# Autodesk Inventor assembly: XY_Assemblie
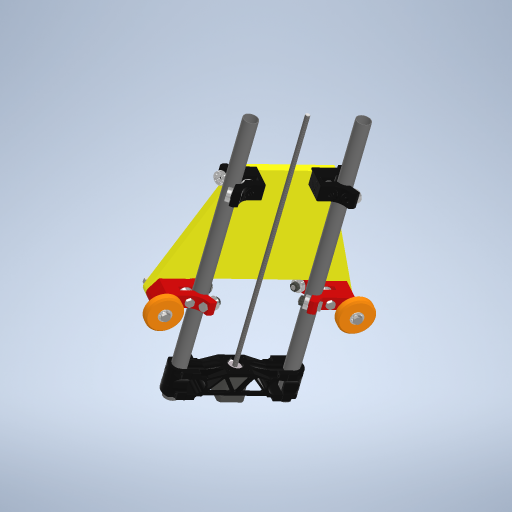
[picture p0: Inventor's stored thumbnail of the model, 512x512]
Saved by Autodesk Inventor 2023 (Build 270158000, 158)
## iProperties
Created: 2023-11-24
Part Number: XY_Assemblie
Document SubType Name: Assembly
Designer: danie
Author: danie
## Documents named in this file (14)
- D:\Diplomarbeit\3d-model\basis_roboter\low_rider_v2\custom_files\XY_Assemblie.iam
- D:\Diplomarbeit\3d-model\basis_roboter\low_rider_v2\custom_files\XZ.ipt
- D:\Diplomarbeit\3d-model\basis_roboter\low_rider_v2\custom_files\XZ_Pipe.ipt
- D:\Diplomarbeit\3d-model\basis_roboter\low_rider_v2\custom_files\XZ_Main.ipt
- D:\Diplomarbeit\3d-model\basis_roboter\low_rider_v2\custom_files\Lower_Za.ipt
- D:\Diplomarbeit\3d-model\basis_roboter\low_rider_v2\custom_files\Lower_Zb.ipt
- D:\Diplomarbeit\3d-model\basis_roboter\low_rider_v2\custom_files\Bearing.ipt
- D:\Diplomarbeit\3d-model\basis_roboter\low_rider_v2\custom_files\XY_Plate_.ipt
- D:\Diplomarbeit\3d-model\basis_roboter\low_rider_v2\custom_files\YZ_Roller_Assemblie.iam
- D:\Diplomarbeit\3d-model\basis_roboter\low_rider_v2\custom_files\Wheel_Assemblie.iam
- C:\Users\danie\OneDrive\Documents\Inventor\Content Center Files\R2023\en-US\AS 1111\AS 1111 - M8 x 70.ipt
- C:\Users\danie\OneDrive\Documents\Inventor\Content Center Files\R2023\en-US\ISO 4032(2)\ISO 4032 - M8 - ISO.ipt
- C:\Users\danie\OneDrive\Documents\Inventor\Content Center Files\R2023\en-US\AS 1111\AS 1111 - M8 x 90.ipt
- D:\Diplomarbeit\3d-model\basis_roboter\nema 17\dle-la-0003_01.ipt
## Components (31 placed, 13 different names)
1. XZ:1 — Rigid:20, Rigid:25
2. XZ_Pipe:1 — Rigid:25
3. XZ:2 — Rigid:19, Rigid:24
4. XZ_Pipe:2 — Rigid:24
5. XZ_Main:1 — Rigid:19, Rigid:20, Mate:17, Mate:19, Angle:3, Rigid:26
6. Lower_Za:1 — Rotational:3, Rotational:4, Rotational:5, Rigid:12
7. Lower_Zb:1 — Rotational:1, Rotational:2, Rigid:5, Rigid:13
8. Bearing:1 — Rotational:2
9. Bearing:2 — Rigid:5
10. Bearing:3 — Rotational:1
11. Bearing:4 — Rotational:3
12. Bearing:5 — Rotational:4
13. Bearing:6 — Rotational:5
14. XY_Plate_:1 — Rigid:12, Rigid:13, Angle:1, Rigid:22, Rigid:23, Mate:4, Mate:8, Mate:12, Mate:16, Mate:17, Mate:18, Angle:2
15. YZ_Roller_Assemblie:1 [sub-assembly] — Rigid:22, Mate:1, Mate:2, Mate:3, Rotational:15
16. YZ_Roller_Assemblie:2 [sub-assembly] — Rigid:23, Rotational:14, Mate:5, Mate:6, Mate:7
17. Wheel_Assemblie:1 [sub-assembly] — Rotational:15, Mate:9, Mate:10, Mate:11
18. Wheel_Assemblie:2 [sub-assembly] — Rotational:14, Mate:13, Mate:14, Mate:15
19. AS 1111 - Metric M8 x 70:1 — Mate:1, Mate:2
20. ISO 4032 M8:1 — Mate:3, Mate:4, Insert:1
21. ISO 4032 M8:2 — Insert:1
22. AS 1111 - Metric M8 x 70:2 — Mate:5, Mate:6
23. ISO 4032 M8:3 — Mate:7, Mate:8, Insert:2
24. ISO 4032 M8:4 — Insert:2
25. AS 1111 - Metric M8 x 90:1 — Mate:9, Mate:10
26. ISO 4032 M8:5 — Mate:11, Mate:12, Insert:3
27. ISO 4032 M8:6 — Insert:3
28. AS 1111 - Metric M8 x 90:2 — Mate:13, Mate:14
29. ISO 4032 M8:7 — Mate:15, Mate:16, Insert:4
30. ISO 4032 M8:8 — Insert:4
31. dle-la-0003_01:1 — Rigid:26
## Relationships (44: Mate 20, WeldJoint 10, RevoluteJoint 7, Insert 4, Angle 3)
- Rotational:1 [RevoluteJoint]: Lower_Zb:1 ↔ Bearing:3
- Rotational:2 [RevoluteJoint]: Lower_Zb:1 ↔ Bearing:1
- Rigid:5 [WeldJoint]: Lower_Zb:1 ↔ Bearing:2
- Rotational:3 [RevoluteJoint]: Lower_Za:1 ↔ Bearing:4
- Rotational:4 [RevoluteJoint]: Lower_Za:1 ↔ Bearing:5
- Rotational:5 [RevoluteJoint]: Lower_Za:1 ↔ Bearing:6
- Rigid:12 [WeldJoint]: Lower_Za:1 ↔ XY_Plate_:1
- Rigid:13 [WeldJoint]: Lower_Zb:1 ↔ XY_Plate_:1
- Rigid:19 [WeldJoint]: XZ:2 ↔ XZ_Main:1
- Rigid:20 [WeldJoint]: XZ:1 ↔ XZ_Main:1
- Angle:1 (0 deg): XY_Plate_:1
- Rigid:22 [WeldJoint]: XY_Plate_:1 ↔ YZ_Roller_Assemblie:1
- Rigid:23 [WeldJoint]: XY_Plate_:1 ↔ YZ_Roller_Assemblie:2
- Rotational:14 [RevoluteJoint]: YZ_Roller_Assemblie:2 ↔ Wheel_Assemblie:2
- Mate:1: YZ_Roller_Assemblie:1 ↔ AS 1111 - Metric M8 x 70:1
- Mate:2: YZ_Roller_Assemblie:1 ↔ AS 1111 - Metric M8 x 70:1
- Mate:3: YZ_Roller_Assemblie:1 ↔ ISO 4032 M8:1
- Mate:4: XY_Plate_:1 ↔ ISO 4032 M8:1
- Insert:1: ISO 4032 M8:1 ↔ ISO 4032 M8:2
- Mate:5: YZ_Roller_Assemblie:2 ↔ AS 1111 - Metric M8 x 70:2
- Mate:6: YZ_Roller_Assemblie:2 ↔ AS 1111 - Metric M8 x 70:2
- Mate:7: YZ_Roller_Assemblie:2 ↔ ISO 4032 M8:3
- Mate:8: XY_Plate_:1 ↔ ISO 4032 M8:3
- Insert:2: ISO 4032 M8:3 ↔ ISO 4032 M8:4
- Rotational:15 [RevoluteJoint]: YZ_Roller_Assemblie:1 ↔ Wheel_Assemblie:1
- Mate:9: Wheel_Assemblie:1 ↔ AS 1111 - Metric M8 x 90:1
- Mate:10: Wheel_Assemblie:1 ↔ AS 1111 - Metric M8 x 90:1
- Mate:11: Wheel_Assemblie:1 ↔ ISO 4032 M8:5
- Mate:12: XY_Plate_:1 ↔ ISO 4032 M8:5
- Insert:3: ISO 4032 M8:5 ↔ ISO 4032 M8:6
- Mate:13: Wheel_Assemblie:2 ↔ AS 1111 - Metric M8 x 90:2
- Mate:14: Wheel_Assemblie:2 ↔ AS 1111 - Metric M8 x 90:2
- Mate:15: Wheel_Assemblie:2 ↔ ISO 4032 M8:7
- Mate:16: XY_Plate_:1 ↔ ISO 4032 M8:7
- Insert:4: ISO 4032 M8:7 ↔ ISO 4032 M8:8
- Mate:17: XZ_Main:1 ↔ XY_Plate_:1
- Mate:18: XY_Plate_:1
- Angle:2 (0 deg): XY_Plate_:1
- Mate:19: XZ_Main:1
- Angle:3 (0 deg): XZ_Main:1
- Mate:20
- Rigid:24 [WeldJoint] (10 mm): XZ:2 ↔ XZ_Pipe:2
- Rigid:25 [WeldJoint] (10 mm): XZ:1 ↔ XZ_Pipe:1
- Rigid:26 [WeldJoint]: XZ_Main:1 ↔ dle-la-0003_01:1
